# Autodesk Inventor assembly: bmx_arm.v1
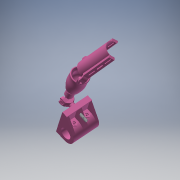
[picture p0: Inventor's stored thumbnail of the model, 180x180]
Saved by Autodesk Inventor 2016 (Build 200138000, 138)
## iProperties
Created: 2015-10-04
Part Number: bmx_arm.v1
Document SubType Name: Assembly
Designer: eedoga
Author: eedoga
## Documents named in this file (9)
- X:\GitHub Repos\BMXArm-MyContribution\bmx_arm.iam
- X:\GitHub Repos\BMXArm-MyContribution\wrist-base1.ipt
- X:\GitHub Repos\BMXArm-MyContribution\wrist-forearm.ipt
- X:\GitHub Repos\BMXArm-MyContribution\carbon-fiber-forearm.ipt
- X:\GitHub Repos\BMXArm-MyContribution\pin.ipt
- X:\GitHub Repos\BMXArm-MyContribution\bike_gipper.ipt
- X:\GitHub Repos\BMXArm-MyContribution\Hair Pin Cotter Pin.ipt
- X:\GitHub Repos\BMXArm-MyContribution\BMX-forearm.ipt
- X:\GitHub Repos\BMXArm-MyContribution\rit-triceps.ipt
## Components (8 placed, 8 different names)
1. wrist-base1:2 — Mate:4, Flush:12, Mate:6, Mate:7
2. wrist-forearm:2 — Mate:4, Flush:12, Flush:13, Mate:5, Angle:3, Flush:14
3. carbon-fiber-forearm:1 — Flush:13, Rotational:1
4. pin:1 — Mate:6, Mate:7, Mate:8, Mate:9, Rotation/Translation:1
5. bike_gipper:1 — Mate:8, Rotation/Translation:1
6. Hair Pin Cotter Pin:1 — Mate:9
7. BMX-forearm:1 — Rotational:1, Rotational:2
8. rit-triceps:1 — Rotational:2
## Relationships (13: Mate 6, Flush 3, RevoluteJoint 2, Angle 1, RelateRotateTranslate 1)
- Mate:4: wrist-base1:2 ↔ wrist-forearm:2
- Flush:12 (-0.1524 mm): wrist-base1:2 ↔ wrist-forearm:2
- Flush:13: wrist-forearm:2 ↔ carbon-fiber-forearm:1
- Mate:5: wrist-forearm:2
- Angle:3 (330 deg): wrist-forearm:2
- Flush:14: wrist-forearm:2
- Mate:6: wrist-base1:2 ↔ pin:1
- Mate:7: wrist-base1:2 ↔ pin:1
- Mate:8: pin:1 ↔ bike_gipper:1
- Mate:9: pin:1 ↔ Hair Pin Cotter Pin:1
- Rotation/Translation:1 [RelateRotateTranslate] (39.9034 mm): pin:1 ↔ bike_gipper:1
- Rotational:1 [RevoluteJoint]: carbon-fiber-forearm:1 ↔ BMX-forearm:1
- Rotational:2 [RevoluteJoint] (-1.27 mm): BMX-forearm:1 ↔ rit-triceps:1
